# Autodesk Inventor assembly: Ensamblaje vacuometro
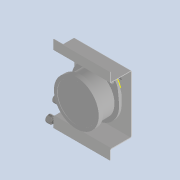
[picture p0: Inventor's stored thumbnail of the model, 180x180]
Saved by Autodesk Inventor 2021 (Build 250183000, 183)
## iProperties
Created: 2021-06-01
Part Number: Ensamblaje vacuometro
Document SubType Name: Assembly
Designer: Admin
Author: Admin
## Documents named in this file (4)
- E:\Documentos\Documentos\Michael_Rodriguez\Universidad_Nacional\Doceaba matricula\PAI\Proyecto PAI\Proyecto_PAI_2021\01 CAD\Ensamblaje vacuometro.iam
- C:\Users\Admin\Documents\Inventor\Content Center Files\R2021\es-ES\BS 4168(1)\BS 4168 - M4 x 20(1).ipt
- E:\Documentos\Documentos\Michael_Rodriguez\Universidad_Nacional\Doceaba matricula\PAI\Proyecto PAI\Proyecto_PAI_2021\01 CAD\Base vacuometro.ipt
- E:\Documentos\Documentos\Michael_Rodriguez\Universidad_Nacional\Doceaba matricula\PAI\Proyecto PAI\Proyecto_PAI_2021\01 CAD\Vacuometro.ipt
## Components (4 placed, 3 different names)
1. BS 4168 : Pieza 1 Tornillo de cabeza cilíndrica con hueco hexagonal - Métrico M4 x 20:1
2. BS 4168 : Pieza 1 Tornillo de cabeza cilíndrica con hueco hexagonal - Métrico M4 x 20:2
3. Base vacuometro:1 — Coincidencia:1, Coincidencia:2, Coincidencia:3
4. Vacuometro:1 — Coincidencia:1, Coincidencia:2, Coincidencia:3
## Relationships (3: Mate 3)
- Coincidencia:1 [Mate]: Base vacuometro:1 ↔ Vacuometro:1
- Coincidencia:2 [Mate]: Base vacuometro:1 ↔ Vacuometro:1
- Coincidencia:3 [Mate]: Base vacuometro:1 ↔ Vacuometro:1
